# Autodesk Inventor assembly: half_motor_driven_shaft
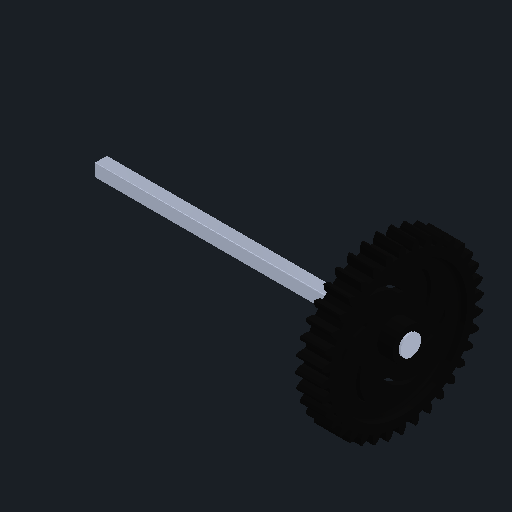
[picture p0: Inventor's stored thumbnail of the model, 512x512]
Saved by Autodesk Inventor 2025 (Build 290162000, 162)
## iProperties
Created: 2024-08-22
Part Number: half_motor_driven_shaft
Document SubType Name: Assembly
Designer: averey
Author: averey
## Documents named in this file (6)
- D:\vex_robotics_high_stakes\hardware\cad\bots\ENIGMA\chassis\drivetrain\drivebay\half_motor_driven_shaft.iam
- D:\vex_robotics_high_stakes\hardware\cad\VEX-CAD-Inventor\Motion\Gears\LS 36T Gear.ipt
- D:\vex_robotics_high_stakes\hardware\cad\VEX-CAD-Inventor\Motion\Shaft LS\Shaft LS Capped\Shaft LS Capped 3.0.ipt
- C:\Users\avere\vex_robotics_high_stakes\hardware\cad\VEX-CAD-Inventor\Motion\Shaft LS\Shaft LS Capped.ipt
- D:\vex_robotics_high_stakes\hardware\cad\VEX-CAD-Inventor\Motion\Spacers\Spacer Nylon .375 OD\NSpacer .375 OD x .125.ipt
- C:\Users\avere\vex_robotics_high_stakes\hardware\cad\VEX-CAD-Inventor\Motion\Spacers\Spacer Nylon .375 OD.ipt
## Components (3 placed, 3 different names)
1. LS 36T Gear:1 — Insert:2
2. Shaft LS Capped 3.0:1
3. NSpacer .375 OD x .125:1 — Insert:2
## Relationships (2: Insert 2)
- [Insert]: LS 36T Gear:1 ↔ Shaft LS Capped 3.0:1
- Insert:2: LS 36T Gear:1 ↔ NSpacer .375 OD x .125:1
